# Autodesk Inventor assembly: testassembly
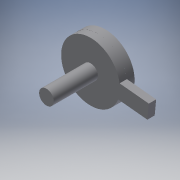
[picture p0: Inventor's stored thumbnail of the model, 180x180]
Saved by Autodesk Inventor 2016 (Build 200138000, 138)
## iProperties
Created: 2015-12-12
Part Number: testassembly
Document SubType Name: Assembly
Designer: Louis
Author: Louis
## Documents named in this file (3)
- C:\Users\Louis\Desktop\Random Stuff\testcadstuff\testassembly.iam
- C:\Users\Louis\Desktop\Random Stuff\testcadstuff\holder.ipt
- C:\Users\Louis\Desktop\Random Stuff\testcadstuff\spinnything.ipt
## Components (2 placed, 2 different names)
1. holder:1 — Mate:1, Mate:2
2. spinnything:1 — Mate:1, Mate:2
## Relationships (2: Mate 2)
- Mate:1: holder:1 ↔ spinnything:1
- Mate:2: holder:1 ↔ spinnything:1
